# Autodesk Inventor assembly: Ensamblaje_Robot_Semillero.iam_V2.0
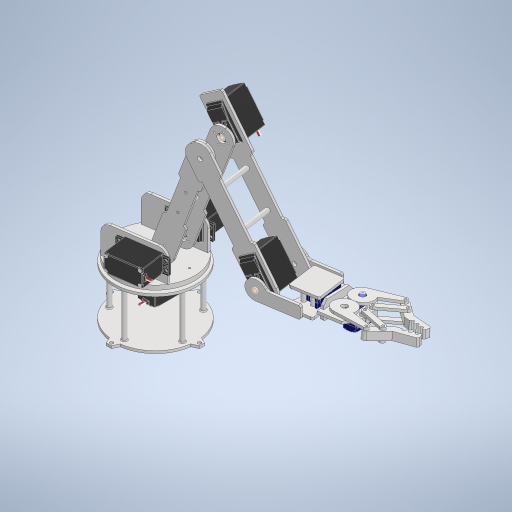
[picture p0: Inventor's stored thumbnail of the model, 512x512]
Saved by Autodesk Inventor 2023 (Build 270158000, 158)
## iProperties
Created: 2024-10-03
Part Number: Ensamblaje_Robot_Semillero.iam_V2.0
Document SubType Name: Assembly
Designer: sebas
Author: sebas
## Documents named in this file (7)
- C:\Users\sebas\OneDrive\Documentos\ILLERO_MODELADO_ROBOT\Ensamblaje_Robot_Semillero.iam_V2.0.iam
- C:\Users\sebas\OneDrive\Documentos\ILLERO_MODELADO_ROBOT\Ensamble_1.iam
- C:\Users\sebas\OneDrive\Documentos\ILLERO_MODELADO_ROBOT\Ensamble_2.iam
- C:\Users\sebas\OneDrive\Documentos\ILLERO_MODELADO_ROBOT\Ensamble_4.iam
- C:\Users\sebas\OneDrive\Documentos\ILLERO_MODELADO_ROBOT\Ensamble_5.iam
- C:\Users\sebas\OneDrive\Documentos\ILLERO_MODELADO_ROBOT\Ensamble_6_Pinza.iam
- C:\Users\sebas\OneDrive\Documentos\ILLERO_MODELADO_ROBOT\Ensamblaje_3.iam
## Components (6 placed, 6 different names)
1. Ensamble_1:1 [sub-assembly] — Coincidencia:1, Coincidencia:2, Coincidencia:3, Coincidencia:4
2. Ensamble_2:1 [sub-assembly] — Coincidencia:3, Coincidencia:4, Coincidencia:5, Coincidencia:6
3. Ensamblaje_3:1 [sub-assembly] — Coincidencia:5, Coincidencia:6, Coincidencia:7, Coincidencia:8
4. Ensamble_4:1 [sub-assembly] — Coincidencia:7, Coincidencia:8, Coincidencia:9, Coincidencia:10
5. Ensamble_5:1 [sub-assembly] — Coincidencia:9, Coincidencia:10, Coincidencia:11, Coincidencia:12
6. Ensamble_6_Pinza:1 [sub-assembly] — Coincidencia:11, Coincidencia:12
## Relationships (12: Mate 12)
- Coincidencia:1 [Mate]: Ensamble_1:1
- Coincidencia:2 [Mate]: Ensamble_1:1
- Coincidencia:3 [Mate] (2 mm): Ensamble_1:1 ↔ Ensamble_2:1
- Coincidencia:4 [Mate]: Ensamble_1:1 ↔ Ensamble_2:1
- Coincidencia:5 [Mate]: Ensamble_2:1 ↔ Ensamblaje_3:1
- Coincidencia:6 [Mate] (6 mm): Ensamble_2:1 ↔ Ensamblaje_3:1
- Coincidencia:7 [Mate]: Ensamblaje_3:1 ↔ Ensamble_4:1
- Coincidencia:8 [Mate] (4 mm): Ensamblaje_3:1 ↔ Ensamble_4:1
- Coincidencia:9 [Mate]: Ensamble_4:1 ↔ Ensamble_5:1
- Coincidencia:10 [Mate] (2 mm): Ensamble_4:1 ↔ Ensamble_5:1
- Coincidencia:11 [Mate]: Ensamble_5:1 ↔ Ensamble_6_Pinza:1
- Coincidencia:12 [Mate]: Ensamble_5:1 ↔ Ensamble_6_Pinza:1
